# Autodesk Inventor assembly: КВ33.044.100 - Блок управления
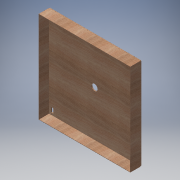
[picture p0: Inventor's stored thumbnail of the model, 180x180]
Saved by Autodesk Inventor 2019 (Build 230136000, 136)
## iProperties
Created: 2019-08-10
Part Number: КВ33.044.100 - Блок управления
Material: Типовые
Document SubType Name: Assembly
Designer: Петров Иван
Author: Петров Иван
## Documents named in this file (3)
- E:\IVAN\Kvantoriada2019\optimal_gripper\hardware\КВ33.044.100 - Блок управления.iam
- E:\IVAN\Kvantoriada2019\optimal_gripper\hardware\КВ33.044.002 - Дно блока управления.ipt
- E:\IVAN\Kvantoriada2019\optimal_gripper\hardware\КВ33.044.004 - Стенка блока управления.ipt
## Components (5 placed, 2 different names)
1. КВ33.044.002 - Дно блока управления:1 — Совмещение:1, Совмещение:2, Совмещение:3, Совмещение:4, Совмещение:5, Совмещение:6, Совмещение:7, Совмещение:8, Совмещение:9, Совмещение:10, Совмещение:11, Совмещение:12
2. КВ33.044.004 - Стенка блока управления:1 — Совмещение:4, Совмещение:5, Совмещение:6
3. КВ33.044.004 - Стенка блока управления:2 — Совмещение:10, Совмещение:11, Совмещение:12
4. КВ33.044.004 - Стенка блока управления:3 — Совмещение:7, Совмещение:8, Совмещение:9
5. КВ33.044.004 - Стенка блока управления:4 — Совмещение:1, Совмещение:2, Совмещение:3
## Relationships (12: Mate 12)
- Совмещение:1 [Mate]: КВ33.044.002 - Дно блока управления:1 ↔ КВ33.044.004 - Стенка блока управления:4
- Совмещение:2 [Mate]: КВ33.044.002 - Дно блока управления:1 ↔ КВ33.044.004 - Стенка блока управления:4
- Совмещение:3 [Mate]: КВ33.044.002 - Дно блока управления:1 ↔ КВ33.044.004 - Стенка блока управления:4
- Совмещение:4 [Mate]: КВ33.044.002 - Дно блока управления:1 ↔ КВ33.044.004 - Стенка блока управления:1
- Совмещение:5 [Mate]: КВ33.044.002 - Дно блока управления:1 ↔ КВ33.044.004 - Стенка блока управления:1
- Совмещение:6 [Mate]: КВ33.044.002 - Дно блока управления:1 ↔ КВ33.044.004 - Стенка блока управления:1
- Совмещение:7 [Mate]: КВ33.044.002 - Дно блока управления:1 ↔ КВ33.044.004 - Стенка блока управления:3
- Совмещение:8 [Mate]: КВ33.044.002 - Дно блока управления:1 ↔ КВ33.044.004 - Стенка блока управления:3
- Совмещение:9 [Mate]: КВ33.044.002 - Дно блока управления:1 ↔ КВ33.044.004 - Стенка блока управления:3
- Совмещение:10 [Mate]: КВ33.044.002 - Дно блока управления:1 ↔ КВ33.044.004 - Стенка блока управления:2
- Совмещение:11 [Mate]: КВ33.044.002 - Дно блока управления:1 ↔ КВ33.044.004 - Стенка блока управления:2
- Совмещение:12 [Mate]: КВ33.044.002 - Дно блока управления:1 ↔ КВ33.044.004 - Стенка блока управления:2
